# Autodesk Inventor assembly: Body Chassis Assembly
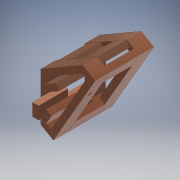
[picture p0: Inventor's stored thumbnail of the model, 180x180]
Saved by Autodesk Inventor 2017 (Build 210142000, 142)
## iProperties
Created: 2018-10-18
Part Number: Body Chassis Assembly
Document SubType Name: Assembly
Designer: Dell
Author: Dell
## Documents named in this file (8)
- C:\Users\Dell\Documents\GitHub\tr2\Body\Body Chassis Assembly.iam
- C:\Users\Dell\Documents\GitHub\tr2\Body\BO03.ipt
- C:\Users\Dell\Documents\GitHub\tr2\Body\BO14.ipt
- C:\Users\Dell\Documents\GitHub\tr2\Body\BO15.ipt
- C:\Users\Dell\Documents\GitHub\tr2\Base\BA07.ipt
- C:\Users\Dell\Documents\GitHub\tr2\Base\BA23.ipt
- C:\Users\Dell\Documents\GitHub\tr2\Body\BO18.ipt
- C:\Users\Dell\Documents\GitHub\tr2\Body\BO19.ipt
## Components (19 placed, 7 different names)
1. BO03:2 — Flush:24, Mate:17, Mate:25, Flush:29, Flush:30, Flush:31, Flush:34, Flush:35, Mate:27, Mate:52
2. BO14:1 — Flush:27, Flush:28, Mate:24, Flush:31, Mate:26, Flush:32, Flush:33, Mate:50, Flush:51, Mate:51, Flush:53
3. BO15:1 — Flush:24, Mate:17
4. BO15:2 — Mate:47, Flush:50, Mate:48
5. BO15:3 — Mate:46, Flush:49, Mate:49
6. BA07:1 — Flush:27, Flush:28, Mate:24, Mate:30, Flush:39, Mate:31, Mate:44, Flush:52
7. BA07:2 — Mate:25, Flush:29, Flush:30, Mate:34, Flush:41, Mate:35
8. BA07:3 — Mate:26, Flush:32, Flush:33, Mate:40, Flush:54
9. BA07:4 — Flush:34, Flush:35, Mate:27, Mate:37
10. BO18:1 — Mate:30, Flush:39, Mate:31, Mate:32, Flush:40, Mate:33, Flush:48, Mate:42, Mate:43
11. BO18:2 — Mate:32, Flush:40, Mate:33, Flush:46
12. BO18:3 — Mate:34, Flush:41, Mate:35, Mate:36, Flush:42, Flush:47, Mate:47, Flush:50
13. BO18:4 — Mate:36, Flush:42, Mate:37, Mate:39, Flush:45, Mate:41, Mate:46, Flush:49
14. BA23:3 — Mate:39, Flush:45, Mate:40
15. BA23:4 — Mate:41, Flush:46, Mate:45, Mate:49
16. BA23:5 — Flush:47, Mate:42, Mate:45, Mate:48
17. BA23:6 — Flush:48, Mate:43, Mate:44
18. BO19:1 — Mate:50, Flush:51, Flush:52, Mate:52
19. BO19:2 — Mate:51, Flush:53, Flush:54
## Relationships (51: Mate 27, Flush 24)
- Flush:24: BO03:2 ↔ BO15:1
- Mate:17: BO03:2 ↔ BO15:1
- Flush:27: BO14:1 ↔ BA07:1
- Flush:28: BO14:1 ↔ BA07:1
- Mate:24: BO14:1 ↔ BA07:1
- Mate:25: BO03:2 ↔ BA07:2
- Flush:29: BO03:2 ↔ BA07:2
- Flush:30: BO03:2 ↔ BA07:2
- Flush:31: BO03:2 ↔ BO14:1
- Mate:26: BO14:1 ↔ BA07:3
- Flush:32: BO14:1 ↔ BA07:3
- Flush:33: BO14:1 ↔ BA07:3
- Flush:34: BO03:2 ↔ BA07:4
- Flush:35: BO03:2 ↔ BA07:4
- Mate:27: BO03:2 ↔ BA07:4
- Mate:30: BA07:1 ↔ BO18:1
- Flush:39: BA07:1 ↔ BO18:1
- Mate:31: BA07:1 ↔ BO18:1
- Mate:32: BO18:1 ↔ BO18:2
- Flush:40: BO18:1 ↔ BO18:2
- Mate:33: BO18:1 ↔ BO18:2
- Mate:34: BA07:2 ↔ BO18:3
- Flush:41: BA07:2 ↔ BO18:3
- Mate:35: BA07:2 ↔ BO18:3
- Mate:36: BO18:3 ↔ BO18:4
- Flush:42: BO18:3 ↔ BO18:4
- Mate:37: BA07:4 ↔ BO18:4
- Mate:39: BO18:4 ↔ BA23:3
- Flush:45: BO18:4 ↔ BA23:3
- Mate:40: BA07:3 ↔ BA23:3
- Mate:41: BO18:4 ↔ BA23:4
- Flush:46: BO18:2 ↔ BA23:4
- Flush:47: BO18:3 ↔ BA23:5
- Flush:48: BO18:1 ↔ BA23:6
- Mate:42: BO18:1 ↔ BA23:5
- Mate:43: BO18:1 ↔ BA23:6
- Mate:44: BA07:1 ↔ BA23:6
- Mate:45: BA23:4 ↔ BA23:5
- Mate:46: BO15:3 ↔ BO18:4
- Mate:47: BO15:2 ↔ BO18:3
- Flush:49: BO15:3 ↔ BO18:4
- Flush:50: BO15:2 ↔ BO18:3
- Mate:48: BO15:2 ↔ BA23:5
- Mate:49: BO15:3 ↔ BA23:4
- Mate:50: BO14:1 ↔ BO19:1
- Flush:51: BO14:1 ↔ BO19:1
- Flush:52: BA07:1 ↔ BO19:1
- Mate:51: BO14:1 ↔ BO19:2
- Flush:53: BO14:1 ↔ BO19:2
- Flush:54: BA07:3 ↔ BO19:2
- Mate:52: BO03:2 ↔ BO19:1
